# Autodesk Inventor assembly: 05.01.СБ1_CHK
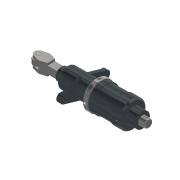
[picture p0: Inventor's stored thumbnail of the model, 180x180]
Saved by Autodesk Inventor 2020.2 (Build 242310000, 310)
## iProperties
Created: 2018-07-09
Part Number: 05.01.СБ1_CHK
Material: Типовые
Description: Амортизатор
Document SubType Name: Assembly
Designer: Сергей
Mass: 2793.56 g
Surface Area: 1144.42 cm^2
Volume: 378.896 cm^3
Density: 7.3729 g/cm^3
Title: 05.01.СБ
Author: MSI-PC
## Documents named in this file (8)
- C:\Users\Сергей\Desktop\Амортизатор_1\05.01.СБ1_CHK.iam
- C:\Users\Сергей\Desktop\Амортизатор_1\05.01.0011_CHK.ipt
- C:\Users\Сергей\Desktop\Амортизатор_1\05.01.0021_CHK.ipt
- C:\Users\Сергей\Desktop\Амортизатор_1\05.01.0031_CHK.ipt
- C:\Users\Сергей\Desktop\Амортизатор_1\05.01.0041_CHK.ipt
- C:\Users\Сергей\Desktop\Амортизатор_1\05.01.0051_CHK.ipt
- C:\Users\Сергей\Desktop\Амортизатор_1\05.01.0061_CHK.ipt
- C:\Users\Сергей\Desktop\Амортизатор_1\05.01.0071_CHK.ipt
## Components (7 placed, 7 different names)
1. 05.01.001:1 — Mate:3, Mate:2, Angle:1, Mate:5, Mate:4
2. 05.01.002:1 — Mate:13, Mate:11, Mate:14, Mate:12
3. 05.01.003:1 — Mate:13, Mate:11, Mate:10, Mate:8, Mate:6
4. 05.01.004:1 — Mate:3, Mate:2, Flush:1, Mate:1
5. 05.01.005:1 — Flush:1, Mate:1
6. 05.01.006:1 — Mate:14, Mate:12, Mate:15, Mate:9
7. 05.01.007:1 — Mate:15, Mate:10, Mate:9, Mate:8, Mate:6, Angle:1, Mate:5, Mate:4
## Relationships (16: Mate 14, Flush 1, Angle 1)
- Mate:13: 05.01.002:1 ↔ 05.01.003:1
- Mate:11: 05.01.002:1 ↔ 05.01.003:1
- Mate:3: 05.01.001:1 ↔ 05.01.004:1
- Mate:2: 05.01.001:1 ↔ 05.01.004:1
- Flush:1: 05.01.004:1 ↔ 05.01.005:1
- Mate:1: 05.01.004:1 ↔ 05.01.005:1
- Mate:14: 05.01.002:1 ↔ 05.01.006:1
- Mate:12: 05.01.002:1 ↔ 05.01.006:1
- Mate:15 (135 mm): 05.01.006:1 ↔ 05.01.007:1
- Mate:10: 05.01.003:1 ↔ 05.01.007:1
- Mate:9: 05.01.006:1 ↔ 05.01.007:1
- Mate:8: 05.01.003:1 ↔ 05.01.007:1
- Mate:6: 05.01.003:1 ↔ 05.01.007:1
- Angle:1 (0 deg): 05.01.001:1 ↔ 05.01.007:1
- Mate:5: 05.01.001:1 ↔ 05.01.007:1
- Mate:4: 05.01.001:1 ↔ 05.01.007:1
